# Autodesk Inventor assembly: camLockMechanism
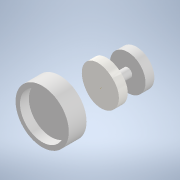
[picture p0: Inventor's stored thumbnail of the model, 180x180]
Saved by Autodesk Inventor 2021.1 (Build 251245000, 245)
## iProperties
Created: 2020-09-02
Part Number: camLockMechanism
Document SubType Name: Assembly
Designer: robst
Author: robst
## Documents named in this file (4)
- C:\git\CAD-Development\robSteele\ShapeWays\TelescopeProjects\TelescopeMount\camLock\camLockMechanism.iam
- C:\git\CAD-Development\robSteele\ShapeWays\TelescopeProjects\TelescopeMount\camLock\Handle.ipt
- C:\git\CAD-Development\robSteele\ShapeWays\TelescopeProjects\TelescopeMount\camLock\Disc Cam1.ipt
- C:\git\CAD-Development\robSteele\ShapeWays\TelescopeProjects\TelescopeMount\camLock\camCircle.ipt
## Components (3 placed, 3 different names)
1. Handle:1 — Mate:1, Mate:2
2. Disc Cam:1 — Mate:1, Mate:2
3. camCircle:1
## Relationships (2: Mate 2)
- Mate:1: Handle:1 ↔ Disc Cam:1
- Mate:2: Handle:1 ↔ Disc Cam:1
